# Autodesk Inventor assembly: rotary encoder_with_knob
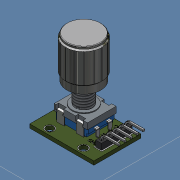
[picture p0: Inventor's stored thumbnail of the model, 180x180]
Saved by Autodesk Inventor 2019 (Build 230136000, 136)
## iProperties
Created: 2019-01-06
Part Number: rotary encoder_with_knob
Material: Generisch
Document SubType Name: Assembly
Designer: Stefan
Mass: 9.41285 g
Surface Area: 56.5564 cm^2
Volume: 4.9702 cm^3
Density: 1.89386 g/cm^3
Author: Stefan
## Documents named in this file (3)
- C:\Users\User\Documents\Inventor\DayLightGlow\Rotary Encoder\rotary encoder_with_knob.iam
- C:\Users\User\Documents\Inventor\DayLightGlow\Rotary Encoder\rotary encoder_chesr_2013.iam
- C:\Users\User\Documents\Inventor\DayLightGlow\Rotary Encoder\knob.ipt
## Components (2 placed, 2 different names)
1. rotary encoder_chesr_2013:1 [sub-assembly] — Passend:1, Fluchtend:1
2. knob:1 — Passend:1, Fluchtend:1
## Relationships (2: Mate 1, Flush 1)
- Passend:1 [Mate]: rotary encoder_chesr_2013:1 ↔ knob:1
- Fluchtend:1 [Flush]: rotary encoder_chesr_2013:1 ↔ knob:1
